# Autodesk Inventor assembly: GearBox Assembly
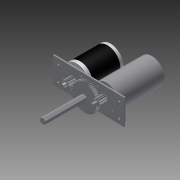
[picture p0: Inventor's stored thumbnail of the model, 180x180]
Saved by Autodesk Inventor 2015 (Build 190159000, 159)
## iProperties
Created: 2015-01-14
Part Number: GearBox Assembly
Document SubType Name: Assembly
Designer: whitaus15
Author: whitaus15
## Documents named in this file (8)
- \\lhssvr02\Homedirs\Robotics Club\CAD Model 2015\GearBox Assembly.iam
- \\lhssvr02\Homedirs\Robotics Club\CAD Model 2015\Imported Components\2014-DiaD-Mecanum\217-3107-001_KEY.ipt
- \\lhssvr02\Homedirs\Robotics Club\CAD Model 2015\Imported Components\2014-DiaD-Mecanum\Mecanum Axle.ipt
- \\lhssvr02\Homedirs\Robotics Club\CAD Model 2015\Imported Components\2014-DiaD-Mecanum\217-2000 - CIM Motor.ipt
- \\lhssvr02\Homedirs\Robotics Club\CAD Model 2015\Parts Folder\Gear Boxes\Imported Components\Toughbox-mini\Toughbox-mini_d02.ipt
- \\lhssvr02\Homedirs\Robotics Club\CAD Model 2015\Parts Folder\Gear Boxes\Imported Components\Toughbox-mini\Toughbox_d06_MIR3.ipt
- \\LHSSVR02\Homedirs\Robotics Club\CAD Model 2015\Parts Folder\Motors\Imported Components\MOT_MiniCIMMotor_217-3371.ipt\MOT_MiniCIMMotor_217-3371.ipt.ipt
- MOT_MiniCIMMotor_217-3371.ipt
## Components (7 placed, 6 different names)
1. 217-3107-001_KEY:1 — Insert:1
2. Mecanum Axle:1 — Flush:1, Mate:1, Mate:2, Mate:3, Mate:4
3. 217-2000 - CIM Motor:1 — Insert:1, Insert:2
4. Toughbox-mini_d02:1 — Flush:1, Insert:2, Mate:4, Mate:5, Mate:6
5. Toughbox_d06_MIR3:1 — Mate:1, Mate:2, Mate:3
6. MOT_MiniCIMMotor_217-3371.ipt:1 — Mate:5, Mate:6, Mate:7
7. 217-3107-001_KEY:2 — Mate:7
## Relationships (10: Mate 7, Insert 2, Flush 1)
- Insert:1 (1.27 mm): 217-3107-001_KEY:1 ↔ 217-2000 - CIM Motor:1
- Flush:1: Mecanum Axle:1 ↔ Toughbox-mini_d02:1
- Insert:2: 217-2000 - CIM Motor:1 ↔ Toughbox-mini_d02:1
- Mate:1: Mecanum Axle:1 ↔ Toughbox_d06_MIR3:1
- Mate:2: Mecanum Axle:1 ↔ Toughbox_d06_MIR3:1
- Mate:3: Mecanum Axle:1 ↔ Toughbox_d06_MIR3:1
- Mate:4: Mecanum Axle:1 ↔ Toughbox-mini_d02:1
- Mate:5: Toughbox-mini_d02:1 ↔ MOT_MiniCIMMotor_217-3371.ipt:1
- Mate:6: Toughbox-mini_d02:1 ↔ MOT_MiniCIMMotor_217-3371.ipt:1
- Mate:7: MOT_MiniCIMMotor_217-3371.ipt:1 ↔ 217-3107-001_KEY:2
